# Autodesk Inventor assembly: Assembly
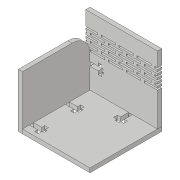
[picture p0: Inventor's stored thumbnail of the model, 180x180]
Saved by Autodesk Inventor 2017 (Build 210142000, 142)
## iProperties
Created: 2019-05-21
Part Number: Assembly
Document SubType Name: Assembly
Designer: markg
Author: markg
## Documents named in this file (4)
- C:\Users\markg\Documents\`School\`ME 433\Assignments&Workspaces\MarkGalperin_ME433_2019\HW13\Autodesk Inventor Files\Assembly.iam
- C:\Users\markg\Documents\`School\`ME 433\Assignments&Workspaces\MarkGalperin_ME433_2019\HW13\Autodesk Inventor Files\base.ipt
- C:\Users\markg\Documents\`School\`ME 433\Assignments&Workspaces\MarkGalperin_ME433_2019\HW13\Autodesk Inventor Files\side1.ipt
- C:\Users\markg\Documents\`School\`ME 433\Assignments&Workspaces\MarkGalperin_ME433_2019\HW13\Autodesk Inventor Files\side2+hinge.ipt
## Components (3 placed, 3 different names)
1. base:1 — Flush:1, Flush:2, Flush:3, Flush:4, Flush:5, Flush:6
2. side1:1 — Flush:1, Flush:2, Flush:3
3. side2+hinge:1 — Flush:4, Flush:5, Flush:6
## Relationships (6: Flush 6)
- Flush:1: base:1 ↔ side1:1
- Flush:2: base:1 ↔ side1:1
- Flush:3: base:1 ↔ side1:1
- Flush:4: base:1 ↔ side2+hinge:1
- Flush:5: base:1 ↔ side2+hinge:1
- Flush:6: base:1 ↔ side2+hinge:1
